# Autodesk Inventor assembly: Base
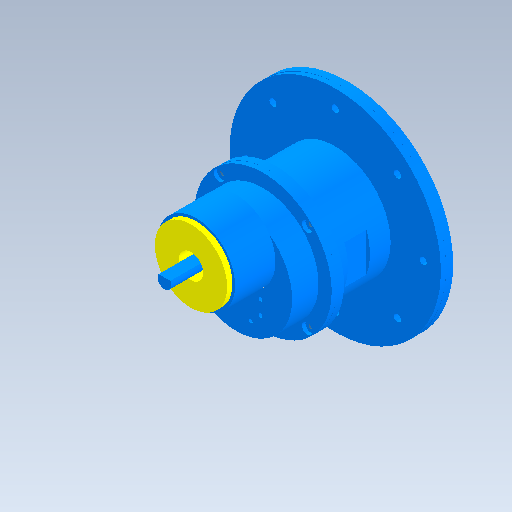
[picture p0: Inventor's stored thumbnail of the model, 512x512]
Saved by Autodesk Inventor 2021 (Build 250183000, 183)
## iProperties
Created: 2022-04-22
Part Number: Base
Document SubType Name: Assembly
Designer: Alcatraz
Author: Alcatraz
## Documents named in this file (7)
- F:\Tesis\TESIS\Matlab\Pruebas\Prueba3_Simulacion2\Base.iam
- F:\Tesis\TESIS\UnionBase.ipt
- F:\Tesis\TESIS\ModuloTrasero_circular4_Parametrizado.ipt
- F:\Tesis\TESIS\AX-12A,18A,12W,MX-12W(stp)\AX-12A.iam
- F:\Tesis\TESIS\ModuloDelantero_Eslabones_3_Parametrizado.ipt
- F:\Tesis\TESIS\Brida_5_parametrizado.ipt
- F:\Tesis\TESIS\rodamiento_dummie.ipt
## Components (7 placed, 6 different names)
1. UnionBase:1 — Coincidencia:1, Coincidencia:2, Coincidencia:3
2. ModuloTrasero_circular4_Parametrizado:1 — Coincidencia:1, Coincidencia:2, Coincidencia:3, Coincidencia:4, Coincidencia:5, Coincidencia:6, Coincidencia:7, Coincidencia:8, Coincidencia:9
3. AX-12A:1 [sub-assembly] — Coincidencia:4, Coincidencia:5, Coincidencia:6, Coincidencia:13, Coincidencia:14, Coincidencia:15
4. ModuloDelantero_Eslabones_3_Parametrizado:1 — Coincidencia:7, Coincidencia:8, Coincidencia:9, Coincidencia:12
5. Brida_5_parametrizado:1 — Coincidencia:13, Coincidencia:14, Coincidencia:15, Coincidencia:16
6. rodamiento_dummie:1 — Coincidencia:10, Coincidencia:11, Coincidencia:12
7. rodamiento_dummie:2 — Coincidencia:10, Coincidencia:11, Coincidencia:16
## Relationships (16: Mate 16)
- Coincidencia:1 [Mate]: UnionBase:1 ↔ ModuloTrasero_circular4_Parametrizado:1
- Coincidencia:2 [Mate]: UnionBase:1 ↔ ModuloTrasero_circular4_Parametrizado:1
- Coincidencia:3 [Mate]: UnionBase:1 ↔ ModuloTrasero_circular4_Parametrizado:1
- Coincidencia:4 [Mate]: ModuloTrasero_circular4_Parametrizado:1 ↔ AX-12A:1
- Coincidencia:5 [Mate]: ModuloTrasero_circular4_Parametrizado:1 ↔ AX-12A:1
- Coincidencia:6 [Mate]: ModuloTrasero_circular4_Parametrizado:1 ↔ AX-12A:1
- Coincidencia:7 [Mate]: ModuloTrasero_circular4_Parametrizado:1 ↔ ModuloDelantero_Eslabones_3_Parametrizado:1
- Coincidencia:8 [Mate]: ModuloTrasero_circular4_Parametrizado:1 ↔ ModuloDelantero_Eslabones_3_Parametrizado:1
- Coincidencia:9 [Mate]: ModuloTrasero_circular4_Parametrizado:1 ↔ ModuloDelantero_Eslabones_3_Parametrizado:1
- Coincidencia:10 [Mate]: rodamiento_dummie:1 ↔ rodamiento_dummie:2
- Coincidencia:11 [Mate]: rodamiento_dummie:1 ↔ rodamiento_dummie:2
- Coincidencia:12 [Mate]: ModuloDelantero_Eslabones_3_Parametrizado:1 ↔ rodamiento_dummie:1
- Coincidencia:13 [Mate]: AX-12A:1 ↔ Brida_5_parametrizado:1
- Coincidencia:14 [Mate]: AX-12A:1 ↔ Brida_5_parametrizado:1
- Coincidencia:15 [Mate]: AX-12A:1 ↔ Brida_5_parametrizado:1
- Coincidencia:16 [Mate]: Brida_5_parametrizado:1 ↔ rodamiento_dummie:2
